# Autodesk Inventor assembly: UHMW
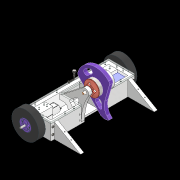
[picture p0: Inventor's stored thumbnail of the model, 180x180]
Saved by Autodesk Inventor 2021 (Build 250183000, 183)
## iProperties
Created: 2021-02-16
Part Number: UHMW
Document SubType Name: Assembly
Designer: Esketitttttt
Mass: 440.061 g
Surface Area: 1342.65 cm^2
Volume: 253.512 cm^3
Density: 1.73586 g/cm^3
Author: Esketitttttt
## Documents named in this file (11)
- C:\Users\Esketitttttt\Documents\GrabCAD\Insomnia 2020\Versions\2 UHMW Mode\UHMW.iam
- C:\Users\Esketitttttt\Documents\GrabCAD\Insomnia 2020\Versions\2 UHMW Mode\AfterComp1ChassisDesigining.ipt
- C:\Users\Esketitttttt\Documents\GrabCAD\Insomnia 2020\Versions\2 UHMW Mode\1ToothNewWeaponAssembly.iam
- C:\Users\Esketitttttt\Documents\GrabCAD\Insomnia 2020\Versions\2 UHMW Mode\WedgeUHMWPiece.ipt
- C:\Users\Esketitttttt\Documents\GrabCAD\Insomnia 2020\Versions\2 UHMW Mode\CorrectSizeWheelsIThink.ipt
- C:\Users\Esketitttttt\Documents\GrabCAD\Insomnia 2020\Versions\2 UHMW Mode\TitaniumWedgeForUhmwVersion.ipt
- C:\Users\Esketitttttt\Documents\GrabCAD\Insomnia 2020\Versions\2 UHMW Mode\90380A011_PHILLIPS THREAD-FORMING SCREW FOR PLASTIC.ipt
- C:\Users\Esketitttttt\Documents\GrabCAD\Insomnia 2020\Versions\2 UHMW Mode\DriveTrainSamdwich.iam
- C:\Users\Esketitttttt\Documents\GrabCAD\Insomnia 2020\Versions\2 UHMW Mode\BatteryMockup.ipt
- C:\Users\Esketitttttt\Documents\GrabCAD\Insomnia 2020\Versions\2 UHMW Mode\AdaptivePrintedLid.ipt
- C:\Users\Esketitttttt\Documents\GrabCAD\Insomnia 2020\Versions\2 UHMW Mode\92400A130_HEX HEAD THREAD-FORMING SCREWS FOR PLASTIC.ipt
## Components (35 placed, 10 different names)
1. AfterComp1ChassisDesigining:1 — Insert:1, Insert:2, Insert:3, Insert:5, Insert:6, Insert:7, Insert:8, Insert:9, Insert:10, Insert:11, Insert:12, Mate:5, Mate:6, Mate:7, Flush:1, Flush:2, Flush:3, Mate:9, Flush:4, Mate:11, Mate:12, Flush:5, Flush:6, Insert:31, Insert:32, Mate:13, Mate:14, Insert:33, Insert:34, Mate:15, Mate:16, Mate:17, Insert:38, Flush:7, Flush:8, Mate:18
2. 1ToothNewWeaponAssembly:1 [sub-assembly] — Mate:18
3. 90380A011_PHILLIPS THREAD-FORMING SCREW FOR PLASTIC:16
4. CorrectSizeWheelsIThink:1 — Insert:34
5. CorrectSizeWheelsIThink:2 — Insert:33
6. DriveTrainSamdwich:1 [sub-assembly] — Insert:31, Mate:14
7. DriveTrainSamdwich:2 [sub-assembly] — Insert:32, Mate:13
8. TitaniumWedgeForUhmwVersion:1 — Insert:35, Insert:36, Insert:37
9. BatteryMockup:1 — Mate:15, Mate:16, Mate:17
10. AdaptivePrintedLid:1 — Flush:7, Flush:8
11. 92400A130_HEX HEAD THREAD-FORMING SCREWS FOR PLASTIC:1
12. 90380A011_PHILLIPS THREAD-FORMING SCREW FOR PLASTIC:2 — Insert:9
13. 90380A011_PHILLIPS THREAD-FORMING SCREW FOR PLASTIC:3 — Insert:10
14. 90380A011_PHILLIPS THREAD-FORMING SCREW FOR PLASTIC:6 — Insert:12
15. 90380A011_PHILLIPS THREAD-FORMING SCREW FOR PLASTIC:7 — Insert:11
16. 90380A011_PHILLIPS THREAD-FORMING SCREW FOR PLASTIC:4 — Insert:7
17. 90380A011_PHILLIPS THREAD-FORMING SCREW FOR PLASTIC:5 — Insert:8
18. 90380A011_PHILLIPS THREAD-FORMING SCREW FOR PLASTIC:8 — Insert:5
19. 90380A011_PHILLIPS THREAD-FORMING SCREW FOR PLASTIC:9 — Insert:6
20. 90380A011_PHILLIPS THREAD-FORMING SCREW FOR PLASTIC:10 — Insert:1
21. 90380A011_PHILLIPS THREAD-FORMING SCREW FOR PLASTIC:11 — Insert:3
22. 90380A011_PHILLIPS THREAD-FORMING SCREW FOR PLASTIC:12 — Insert:38
23. 90380A011_PHILLIPS THREAD-FORMING SCREW FOR PLASTIC:13 — Insert:2
24. WedgeUHMWPiece:1 — Mate:5, Flush:2, Mate:11, Insert:37
25. WedgeUHMWPiece:2 — Mate:6, Flush:3, Mate:12, Insert:35, Insert:36
26. WedgeUHMWPiece:3 — Mate:9, Flush:4, Flush:6
27. WedgeUHMWPiece:4 — Mate:7, Flush:1, Flush:5
28. 90380A011_PHILLIPS THREAD-FORMING SCREW FOR PLASTIC:17
29. 90380A011_PHILLIPS THREAD-FORMING SCREW FOR PLASTIC:18
30. 90380A011_PHILLIPS THREAD-FORMING SCREW FOR PLASTIC:19
31. 90380A011_PHILLIPS THREAD-FORMING SCREW FOR PLASTIC:20
32. 90380A011_PHILLIPS THREAD-FORMING SCREW FOR PLASTIC:21
33. 90380A011_PHILLIPS THREAD-FORMING SCREW FOR PLASTIC:22
34. 90380A011_PHILLIPS THREAD-FORMING SCREW FOR PLASTIC:23
35. 90380A011_PHILLIPS THREAD-FORMING SCREW FOR PLASTIC:24
## Relationships (39: Insert 19, Mate 12, Flush 8)
- Insert:1: AfterComp1ChassisDesigining:1 ↔ 90380A011_PHILLIPS THREAD-FORMING SCREW FOR PLASTIC:10
- Insert:2: AfterComp1ChassisDesigining:1 ↔ 90380A011_PHILLIPS THREAD-FORMING SCREW FOR PLASTIC:13
- Insert:3: AfterComp1ChassisDesigining:1 ↔ 90380A011_PHILLIPS THREAD-FORMING SCREW FOR PLASTIC:11
- Insert:5: AfterComp1ChassisDesigining:1 ↔ 90380A011_PHILLIPS THREAD-FORMING SCREW FOR PLASTIC:8
- Insert:6: AfterComp1ChassisDesigining:1 ↔ 90380A011_PHILLIPS THREAD-FORMING SCREW FOR PLASTIC:9
- Insert:7: AfterComp1ChassisDesigining:1 ↔ 90380A011_PHILLIPS THREAD-FORMING SCREW FOR PLASTIC:4
- Insert:8: AfterComp1ChassisDesigining:1 ↔ 90380A011_PHILLIPS THREAD-FORMING SCREW FOR PLASTIC:5
- Insert:9: AfterComp1ChassisDesigining:1 ↔ 90380A011_PHILLIPS THREAD-FORMING SCREW FOR PLASTIC:2
- Insert:10: AfterComp1ChassisDesigining:1 ↔ 90380A011_PHILLIPS THREAD-FORMING SCREW FOR PLASTIC:3
- Insert:11: AfterComp1ChassisDesigining:1 ↔ 90380A011_PHILLIPS THREAD-FORMING SCREW FOR PLASTIC:7
- Insert:12: AfterComp1ChassisDesigining:1 ↔ 90380A011_PHILLIPS THREAD-FORMING SCREW FOR PLASTIC:6
- Mate:5: AfterComp1ChassisDesigining:1 ↔ WedgeUHMWPiece:1
- Mate:6: AfterComp1ChassisDesigining:1 ↔ WedgeUHMWPiece:2
- Mate:7: AfterComp1ChassisDesigining:1 ↔ WedgeUHMWPiece:4
- Flush:1: AfterComp1ChassisDesigining:1 ↔ WedgeUHMWPiece:4
- Flush:2: AfterComp1ChassisDesigining:1 ↔ WedgeUHMWPiece:1
- Flush:3: AfterComp1ChassisDesigining:1 ↔ WedgeUHMWPiece:2
- Mate:9: AfterComp1ChassisDesigining:1 ↔ WedgeUHMWPiece:3
- Flush:4: AfterComp1ChassisDesigining:1 ↔ WedgeUHMWPiece:3
- Mate:11: AfterComp1ChassisDesigining:1 ↔ WedgeUHMWPiece:1
- Mate:12: AfterComp1ChassisDesigining:1 ↔ WedgeUHMWPiece:2
- Flush:5: AfterComp1ChassisDesigining:1 ↔ WedgeUHMWPiece:4
- Flush:6: AfterComp1ChassisDesigining:1 ↔ WedgeUHMWPiece:3
- Insert:31: AfterComp1ChassisDesigining:1 ↔ DriveTrainSamdwich:1
- Insert:32: AfterComp1ChassisDesigining:1 ↔ DriveTrainSamdwich:2
- Mate:13: AfterComp1ChassisDesigining:1 ↔ DriveTrainSamdwich:2
- Mate:14: AfterComp1ChassisDesigining:1 ↔ DriveTrainSamdwich:1
- Insert:33: AfterComp1ChassisDesigining:1 ↔ CorrectSizeWheelsIThink:2
- Insert:34: AfterComp1ChassisDesigining:1 ↔ CorrectSizeWheelsIThink:1
- Insert:35: TitaniumWedgeForUhmwVersion:1 ↔ WedgeUHMWPiece:2
- Insert:36: TitaniumWedgeForUhmwVersion:1 ↔ WedgeUHMWPiece:2
- Insert:37: TitaniumWedgeForUhmwVersion:1 ↔ WedgeUHMWPiece:1
- Mate:15: AfterComp1ChassisDesigining:1 ↔ BatteryMockup:1
- Mate:16: AfterComp1ChassisDesigining:1 ↔ BatteryMockup:1
- Mate:17 (1.27 mm): AfterComp1ChassisDesigining:1 ↔ BatteryMockup:1
- Insert:38: AfterComp1ChassisDesigining:1 ↔ 90380A011_PHILLIPS THREAD-FORMING SCREW FOR PLASTIC:12
- Flush:7: AfterComp1ChassisDesigining:1 ↔ AdaptivePrintedLid:1
- Flush:8: AfterComp1ChassisDesigining:1 ↔ AdaptivePrintedLid:1
- Mate:18: AfterComp1ChassisDesigining:1 ↔ 1ToothNewWeaponAssembly:1
